# Autodesk Inventor assembly: EL2-CGB-100
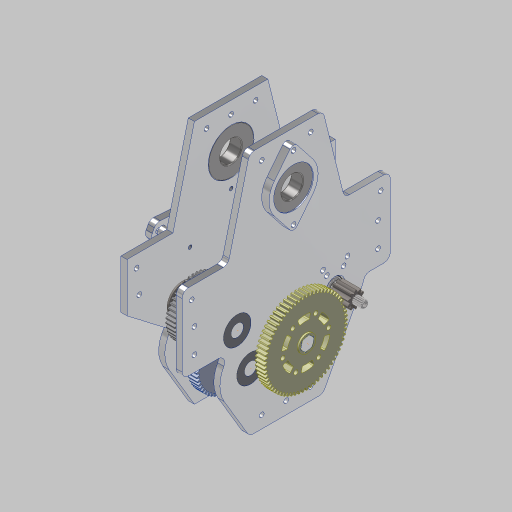
[picture p0: Inventor's stored thumbnail of the model, 512x512]
Saved by Autodesk Inventor 2023.5 (Build 275446000, 446)
## iProperties
Created: 2025-01-19
Part Number: EL2-CGB-100
Document SubType Name: Assembly
Designer: mavericks
Author: mavericks
## Documents named in this file (21)
- C:\Users\slick\OneDrive\Desktop\2025-ReefScape---CAD\Elevator\EL2-CGB\EL2-CGB-100.iam
- C:\Users\slick\OneDrive\Desktop\2025-ReefScape---CAD\Elevator\EL2-CGB\EL2-CGB-001.ipt
- C:\Users\slick\OneDrive\Desktop\2025-ReefScape---CAD\COMMON PARTS\GEARS\20dp .5 hex\50t_Aluminum_Spur_Gear_20_DP_1_2_Hex_Bore_217-3572.ipt
- C:\Users\slick\OneDrive\Desktop\2025-ReefScape---CAD\COMMON PARTS\GEARS\20dp .5 hex\18t_Aluminum_Spur_Gear_20_DP_1_2_Hex_Bore_217-3209.ipt
- C:\Users\slick\OneDrive\Desktop\2025-ReefScape---CAD\COMMON PARTS\BEARINGS\0_875_ID_x_1_875_OD_X_0_500_Radial_Bearing_EE11S-2RS.ipt
- C:\Users\slick\OneDrive\Desktop\2025-ReefScape---CAD\COMMON PARTS\BEARINGS\0_500_ID_x_1_125_OD_x_0_313_WD_Flanged_Bearing_217-2731.ipt
- C:\Users\slick\OneDrive\Desktop\2025-ReefScape---CAD\COMMON PARTS\GEARS\20dp .5 hex\44t_Aluminum_Spur_Gear_20_DP_1_2_Hex_Bore_217-2710.ipt
- C:\Users\slick\OneDrive\Desktop\2025-ReefScape---CAD\COMMON PARTS\GEARS\20dp .5 hex\24t_Aluminum_Spur_Gear_20_DP_1_2_Hex_Bore_217-2704.ipt
- C:\Users\slick\OneDrive\Desktop\2025-ReefScape---CAD\Elevator\EL2-CGB\EL2-CGB-002.ipt
- C:\Users\slick\OneDrive\Desktop\2025-ReefScape---CAD\Elevator\EL2-CGB\EL2-CGB-003.ipt
- C:\Users\slick\OneDrive\Desktop\2025-ReefScape---CAD\Elevator\EL2-CGB\EL2-CGB-004.ipt
- C:\Users\slick\OneDrive\Desktop\2025-ReefScape---CAD\COMMON PARTS\BEARINGS\0_500_Hex_ID_x_1_125_OD_x_0_313_WD_Flanged_Bearing_v2_217-3875.ipt
- C:\Users\slick\OneDrive\Desktop\2025-ReefScape---CAD\COMMON PARTS\GEARS\20dp .5 hex\66t_Aluminum_Spur_Gear_20_DP_1_2_Hex_Bore_VersaKeys_217-3223.ipt
- C:\Users\slick\OneDrive\Desktop\2025-ReefScape---CAD\COMMON PARTS\Z - STEPS\WCP-1008\WCP-1008.ipt
- C:\Users\slick\OneDrive\Desktop\2025-ReefScape---CAD\COMMON PARTS\SPROCKETS\35\12t_Aluminum_Hub_Sprocket_35_Chain_1_2_Hex_Bore_217-2662.ipt
- C:\Users\slick\OneDrive\Desktop\2025-ReefScape---CAD\COMMON PARTS\MOTORS\WCP-0941 x44 Kracken.ipt
- C:\Users\slick\OneDrive\Desktop\2025-ReefScape---CAD\Elevator\EL2-CGB\EL2-CGB-007.ipt
- C:\Users\slick\OneDrive\Desktop\2025-ReefScape---CAD\Elevator\EL2-CGB\EL2-CGB-008.ipt
- C:\Users\slick\OneDrive\Desktop\2025-ReefScape---CAD\Elevator\EL2-CGB\EL2-CGB-010.ipt
- C:\Users\slick\OneDrive\Desktop\2025-ReefScape---CAD\COMMON PARTS\SPROCKETS\35\WCP-0976.ipt
- C:\Users\slick\OneDrive\Desktop\2025-ReefScape---CAD\Elevator\EL2-CGB\EL2-CGB-011.ipt
## Components (31 placed, 20 different names)
1. EL2-CGB-001:1 — Mate:13, Flush:2, Insert:6, Insert:14, Mate:20, Mate:21, Mate:22, Insert:19, Mate:29, Mate:30, Insert:21, Insert:23, Insert:24
2. WCP-0941 x44 Kracken:1 — Mate:28, Mate:29, Mate:30, Insert:21, Mate:31
3. WCP-1008:1 — Mate:28, Mate:31
4. 66t_Aluminum_Spur_Gear_20_DP_1_2_Hex_Bore_VersaKeys_217-3223:1 — Flush:8, Mate:25
5. 50t_Aluminum_Spur_Gear_20_DP_1_2_Hex_Bore_217-3572:1 — Flush:3, Mate:16, Mate:33
6. 24t_Aluminum_Spur_Gear_20_DP_1_2_Hex_Bore_217-2704:1 — Mate:16, Flush:4
7. 18t_Aluminum_Spur_Gear_20_DP_1_2_Hex_Bore_217-3209:1 — Flush:3, Mate:19
8. 44t_Aluminum_Spur_Gear_20_DP_1_2_Hex_Bore_217-2710:1 — Flush:4, Mate:32
9. EL2-CGB-002:1 — Insert:8
10. EL2-CGB-004:1 — Mate:17, Mate:19, Flush:7, Flush:8
11. EL2-CGB-003:1 — Mate:20, Mate:21, Mate:22, Flush:7, Insert:15, Insert:16, Mate:26, Flush:9, Insert:18, Insert:25, Insert:26, Mate:50, Mate:51, Mate:52
12. EL2-CGB-004:2 — Insert:20
13. 12t_Aluminum_Hub_Sprocket_35_Chain_1_2_Hex_Bore_217-2662:1 — Mate:27, Flush:10
14. EL2-CGB-007:1 — Mate:43, Mate:44, Mate:48, Mate:49, Mate:50, Mate:53
15. EL2-CGB-007:2 — Mate:45, Mate:46, Mate:47, Mate:49, Mate:51, Mate:54
16. EL2-CGB-008:1 — Insert:23, Insert:24
17. EL2-CGB-008:2 — Insert:25, Insert:26
18. EL2-CGB-010:1 — Angle:1, Mate:52, Insert:27, Mate:53, Mate:54
19. EL2-CGB-010:3 — Angle:1, Mate:43, Mate:44, Mate:45, Mate:46, Mate:47, Mate:48, Insert:28
20. WCP-0976:1 — Mate:57, Mate:58, Flush:10
21. 0_500_ID_x_1_125_OD_x_0_313_WD_Flanged_Bearing_217-2731:9 — Insert:28, Mate:55
22. 0_500_ID_x_1_125_OD_x_0_313_WD_Flanged_Bearing_217-2731:10 — Insert:27, Mate:55, Insert:29
23. EL2-CGB-011:1 — Insert:29, Mate:57, Mate:58
24. 0_875_ID_x_1_875_OD_X_0_500_Radial_Bearing_EE11S-2RS:1 — Mate:13, Flush:2
25. 0_500_ID_x_1_125_OD_x_0_313_WD_Flanged_Bearing_217-2731:5 — Insert:6, Insert:8, Mate:33
26. 0_500_Hex_ID_x_1_125_OD_x_0_313_WD_Flanged_Bearing_v2_217-3875:1 — Insert:14, Mate:17, Mate:25
27. 0_500_Hex_ID_x_1_125_OD_x_0_313_WD_Flanged_Bearing_v2_217-3875:2 — Insert:18, Mate:27
28. 0_500_ID_x_1_125_OD_x_0_313_WD_Flanged_Bearing_217-2731:6 — Insert:15
29. 0_500_ID_x_1_125_OD_x_0_313_WD_Flanged_Bearing_217-2731:7 — Insert:16
30. 0_875_ID_x_1_875_OD_X_0_500_Radial_Bearing_EE11S-2RS:2 — Mate:26, Flush:9
31. 0_500_ID_x_1_125_OD_x_0_313_WD_Flanged_Bearing_217-2731:8 — Insert:19, Insert:20, Mate:32
## Relationships (56: Mate 32, Insert 16, Flush 7, Angle 1)
- [Mate]: EL2-CGB-001:1 ↔ 24t_Aluminum_Spur_Gear_20_DP_1_2_Hex_Bore_217-2704:1
- Mate:13: EL2-CGB-001:1 ↔ 0_875_ID_x_1_875_OD_X_0_500_Radial_Bearing_EE11S-2RS:1
- Flush:2: EL2-CGB-001:1 ↔ 0_875_ID_x_1_875_OD_X_0_500_Radial_Bearing_EE11S-2RS:1
- Insert:6: EL2-CGB-001:1 ↔ 0_500_ID_x_1_125_OD_x_0_313_WD_Flanged_Bearing_217-2731:5
- Insert:8: EL2-CGB-002:1 ↔ 0_500_ID_x_1_125_OD_x_0_313_WD_Flanged_Bearing_217-2731:5
- Flush:3: 50t_Aluminum_Spur_Gear_20_DP_1_2_Hex_Bore_217-3572:1 ↔ 18t_Aluminum_Spur_Gear_20_DP_1_2_Hex_Bore_217-3209:1
- Mate:16: 50t_Aluminum_Spur_Gear_20_DP_1_2_Hex_Bore_217-3572:1 ↔ 24t_Aluminum_Spur_Gear_20_DP_1_2_Hex_Bore_217-2704:1
- Flush:4: 24t_Aluminum_Spur_Gear_20_DP_1_2_Hex_Bore_217-2704:1 ↔ 44t_Aluminum_Spur_Gear_20_DP_1_2_Hex_Bore_217-2710:1
- Insert:14: EL2-CGB-001:1 ↔ 0_500_Hex_ID_x_1_125_OD_x_0_313_WD_Flanged_Bearing_v2_217-3875:1
- Mate:17: EL2-CGB-004:1 ↔ 0_500_Hex_ID_x_1_125_OD_x_0_313_WD_Flanged_Bearing_v2_217-3875:1
- Mate:19: 18t_Aluminum_Spur_Gear_20_DP_1_2_Hex_Bore_217-3209:1 ↔ EL2-CGB-004:1
- Mate:20 (50.8 mm): EL2-CGB-001:1 ↔ EL2-CGB-003:1
- Mate:21: EL2-CGB-001:1 ↔ EL2-CGB-003:1
- Mate:22: EL2-CGB-001:1 ↔ EL2-CGB-003:1
- Flush:7: EL2-CGB-004:1 ↔ EL2-CGB-003:1
- Flush:8: 66t_Aluminum_Spur_Gear_20_DP_1_2_Hex_Bore_VersaKeys_217-3223:1 ↔ EL2-CGB-004:1
- Mate:25: 66t_Aluminum_Spur_Gear_20_DP_1_2_Hex_Bore_VersaKeys_217-3223:1 ↔ 0_500_Hex_ID_x_1_125_OD_x_0_313_WD_Flanged_Bearing_v2_217-3875:1
- Insert:15: EL2-CGB-003:1 ↔ 0_500_ID_x_1_125_OD_x_0_313_WD_Flanged_Bearing_217-2731:6
- Insert:16: EL2-CGB-003:1 ↔ 0_500_ID_x_1_125_OD_x_0_313_WD_Flanged_Bearing_217-2731:7
- Mate:26: EL2-CGB-003:1 ↔ 0_875_ID_x_1_875_OD_X_0_500_Radial_Bearing_EE11S-2RS:2
- Flush:9: EL2-CGB-003:1 ↔ 0_875_ID_x_1_875_OD_X_0_500_Radial_Bearing_EE11S-2RS:2
- Insert:18: EL2-CGB-003:1 ↔ 0_500_Hex_ID_x_1_125_OD_x_0_313_WD_Flanged_Bearing_v2_217-3875:2
- Insert:19: EL2-CGB-001:1 ↔ 0_500_ID_x_1_125_OD_x_0_313_WD_Flanged_Bearing_217-2731:8
- Insert:20: EL2-CGB-004:2 ↔ 0_500_ID_x_1_125_OD_x_0_313_WD_Flanged_Bearing_217-2731:8
- Mate:27: 12t_Aluminum_Hub_Sprocket_35_Chain_1_2_Hex_Bore_217-2662:1 ↔ 0_500_Hex_ID_x_1_125_OD_x_0_313_WD_Flanged_Bearing_v2_217-3875:2
- Mate:28: WCP-0941 x44 Kracken:1 ↔ WCP-1008:1
- Mate:29: EL2-CGB-001:1 ↔ WCP-0941 x44 Kracken:1
- Mate:30: EL2-CGB-001:1 ↔ WCP-0941 x44 Kracken:1
- Insert:21: EL2-CGB-001:1 ↔ WCP-0941 x44 Kracken:1
- Mate:31 (3.175 mm): WCP-0941 x44 Kracken:1 ↔ WCP-1008:1
- Mate:32: 44t_Aluminum_Spur_Gear_20_DP_1_2_Hex_Bore_217-2710:1 ↔ 0_500_ID_x_1_125_OD_x_0_313_WD_Flanged_Bearing_217-2731:8
- Mate:33: 50t_Aluminum_Spur_Gear_20_DP_1_2_Hex_Bore_217-3572:1 ↔ 0_500_ID_x_1_125_OD_x_0_313_WD_Flanged_Bearing_217-2731:5
- Insert:23: EL2-CGB-001:1 ↔ EL2-CGB-008:1
- Insert:24: EL2-CGB-001:1 ↔ EL2-CGB-008:1
- Insert:25: EL2-CGB-003:1 ↔ EL2-CGB-008:2
- Insert:26: EL2-CGB-003:1 ↔ EL2-CGB-008:2
- Angle:1 (0 deg): EL2-CGB-010:1 ↔ EL2-CGB-010:3
- Mate:43: EL2-CGB-007:1 ↔ EL2-CGB-010:3
- Mate:44: EL2-CGB-007:1 ↔ EL2-CGB-010:3
- Mate:45: EL2-CGB-007:2 ↔ EL2-CGB-010:3
- Mate:46: EL2-CGB-007:2 ↔ EL2-CGB-010:3
- Mate:47: EL2-CGB-007:2 ↔ EL2-CGB-010:3
- Mate:48: EL2-CGB-007:1 ↔ EL2-CGB-010:3
- Mate:49 (56.8579 mm): EL2-CGB-007:1 ↔ EL2-CGB-007:2
- Mate:50: EL2-CGB-003:1 ↔ EL2-CGB-007:1
- Mate:51: EL2-CGB-003:1 ↔ EL2-CGB-007:2
- Mate:52: EL2-CGB-003:1 ↔ EL2-CGB-010:1
- Insert:27: EL2-CGB-010:1 ↔ 0_500_ID_x_1_125_OD_x_0_313_WD_Flanged_Bearing_217-2731:10
- Insert:28: EL2-CGB-010:3 ↔ 0_500_ID_x_1_125_OD_x_0_313_WD_Flanged_Bearing_217-2731:9
- Mate:53: EL2-CGB-007:1 ↔ EL2-CGB-010:1
- Mate:54: EL2-CGB-007:2 ↔ EL2-CGB-010:1
- Mate:55: 0_500_ID_x_1_125_OD_x_0_313_WD_Flanged_Bearing_217-2731:9 ↔ 0_500_ID_x_1_125_OD_x_0_313_WD_Flanged_Bearing_217-2731:10
- Insert:29: 0_500_ID_x_1_125_OD_x_0_313_WD_Flanged_Bearing_217-2731:10 ↔ EL2-CGB-011:1
- Mate:57: WCP-0976:1 ↔ EL2-CGB-011:1
- Mate:58: WCP-0976:1 ↔ EL2-CGB-011:1
- Flush:10: 12t_Aluminum_Hub_Sprocket_35_Chain_1_2_Hex_Bore_217-2662:1 ↔ WCP-0976:1
